# Autodesk Inventor assembly: FloatingBarChair
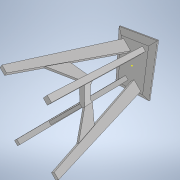
[picture p0: Inventor's stored thumbnail of the model, 180x180]
Saved by Autodesk Inventor 2022 (Build 260153000, 153)
## iProperties
Created: 2021-12-19
Part Number: FloatingBarChair
Document SubType Name: Assembly
Designer: dangl
Author: dangl
## Documents named in this file (8)
- C:\Users\dangl\Documents\WoodWork\FloatingBarChair\FloatingBarChair.iam
- C:\Users\dangl\Documents\WoodWork\FloatingBarChair\ChairTop.ipt
- C:\Users\dangl\Documents\WoodWork\FloatingBarChair\Leg.ipt
- C:\Users\dangl\Documents\WoodWork\FloatingBarChair\LegConnector.ipt
- C:\Users\dangl\Documents\WoodWork\FloatingBarChair\LegConnector_MIR.ipt
- C:\Users\dangl\Documents\WoodWork\FloatingBarChair\LegConnector_MIR1.ipt
- C:\Users\dangl\Documents\WoodWork\FloatingBarChair\LegConnector_MIR_MIR.ipt
- C:\Users\dangl\Documents\WoodWork\FloatingBarChair\LegConnectorBase.ipt
## Components (10 placed, 7 different names)
1. ChairTop:1 — Flush:1, Flush:2, Mate:5, Flush:4, Flush:5, Flush:6
2. Leg:1 — Flush:1, Flush:2, Mate:2, Mate:3, Mate:4, Mate:6, Mate:7, Flush:3
3. Leg:2 — Mate:3, Mate:4
4. Leg:3 — Mate:2, Mate:5
5. Leg:4 — Mate:6, Mate:7
6. LegConnector:1 — Flush:3, Flush:4
7. LegConnector_MIR:1
8. LegConnector_MIR1:1
9. LegConnector_MIR_MIR:1
10. LegConnectorBase:1 — Flush:5, Flush:6
## Relationships (12: Flush 6, Mate 6)
- Flush:1: ChairTop:1 ↔ Leg:1
- Flush:2: ChairTop:1 ↔ Leg:1
- Mate:2: Leg:1 ↔ Leg:3
- Mate:3: Leg:1 ↔ Leg:2
- Mate:4: Leg:1 ↔ Leg:2
- Mate:5: ChairTop:1 ↔ Leg:3
- Mate:6: Leg:1 ↔ Leg:4
- Mate:7: Leg:1 ↔ Leg:4
- Flush:3: Leg:1 ↔ LegConnector:1
- Flush:4: ChairTop:1 ↔ LegConnector:1
- Flush:5: ChairTop:1 ↔ LegConnectorBase:1
- Flush:6: ChairTop:1 ↔ LegConnectorBase:1
